# Autodesk Inventor assembly: DriveRoller
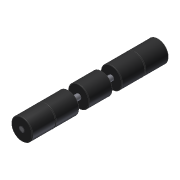
[picture p0: Inventor's stored thumbnail of the model, 180x180]
Saved by Autodesk Inventor 2012 (Build 160160000, 160)
## iProperties
Created: 2012-01-16
Part Number: DriveRoller
Document SubType Name: Assembly
Designer: JesseK
Mass: 204.555 g
Surface Area: 333.257 cm^2
Volume: 142.647 cm^3
Density: 1.43399 g/cm^3
Author: JesseK
## Documents named in this file (3)
- Z:\UserData\Documents\Inventor\team1885frc\Robot2012\Conveyor2\DriveRoller.iam
- Z:\UserData\Documents\Inventor\team1885frc\Robot2012\Conveyor2\RollerAxle.ipt
- Z:\UserData\Documents\Inventor\team1885frc\Robot2012\Conveyor2\Conveyor_Roller_Middle.ipt
## Components (6 placed, 2 different names)
1. RollerAxle:1 — Mate:1, Flush:1, Mate:2, Mate:3, Mate:4, Mate:5
2. Conveyor_Roller_Middle:1 — Mate:1, Flush:1, Mate:6
3. Conveyor_Roller_Middle:2 — Mate:2, Mate:6, Mate:8
4. Conveyor_Roller_Middle:3 — Mate:3
5. Conveyor_Roller_Middle:4 — Mate:4, Mate:7
6. Conveyor_Roller_Middle:5 — Mate:5, Mate:7, Mate:8
## Relationships (9: Mate 8, Flush 1)
- Mate:1: RollerAxle:1 ↔ Conveyor_Roller_Middle:1
- Flush:1: RollerAxle:1 ↔ Conveyor_Roller_Middle:1
- Mate:2: RollerAxle:1 ↔ Conveyor_Roller_Middle:2
- Mate:3: RollerAxle:1 ↔ Conveyor_Roller_Middle:3
- Mate:4: RollerAxle:1 ↔ Conveyor_Roller_Middle:4
- Mate:5: RollerAxle:1 ↔ Conveyor_Roller_Middle:5
- Mate:6: Conveyor_Roller_Middle:1 ↔ Conveyor_Roller_Middle:2
- Mate:7: Conveyor_Roller_Middle:4 ↔ Conveyor_Roller_Middle:5
- Mate:8 (63.5 mm): Conveyor_Roller_Middle:2 ↔ Conveyor_Roller_Middle:5
